# Autodesk Inventor assembly: Level 2
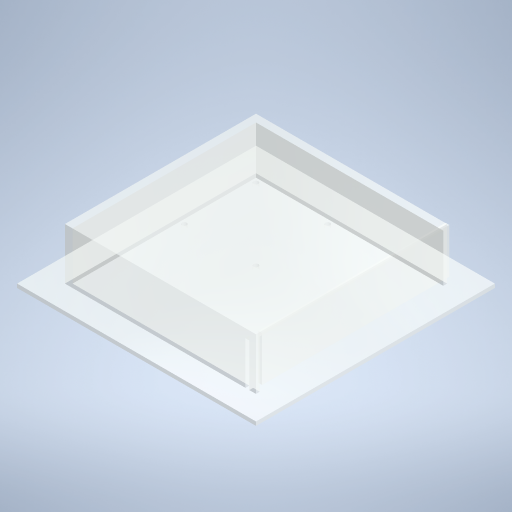
[picture p0: Inventor's stored thumbnail of the model, 512x512]
Saved by Autodesk Inventor 2024 (Build 280153000, 153)
## iProperties
Created: 2023-07-19
Part Number: Level 2
Document SubType Name: Assembly
Designer: javie
Author: javie
## Documents named in this file (3)
- C:\Users\javie\OneDrive\Documents\Inventor\L2\Level 2.iam
- C:\Users\javie\OneDrive\Documents\Inventor\L2\Acrylic Casing.ipt
- C:\Users\javie\OneDrive\Documents\Inventor\L2\Acrylic Top.ipt
## Components (2 placed, 2 different names)
1. Acrylic Casing:1 — Mate:1, Mate:2
2. Acrylic Door:1 — Mate:1, Mate:2
## Relationships (2: Mate 2)
- Mate:1: Acrylic Casing:1 ↔ Acrylic Door:1
- Mate:2: Acrylic Casing:1 ↔ Acrylic Door:1
